# Autodesk Inventor assembly: Shooter-Storage-IntakeAssembly.ver2-1111-2021
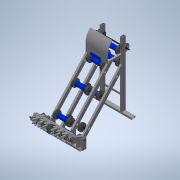
[picture p0: Inventor's stored thumbnail of the model, 180x180]
Saved by Autodesk Inventor 2021 (Build 250183000, 183)
## iProperties
Created: 2020-01-25
Part Number: Shooter-Storage-IntakeAssembly.ver2-1111-2021
Document SubType Name: Assembly
Designer: JMHal
Author: JMHal
## Documents named in this file (6)
- E:\PHRC CADD 2021\PHRC CADD\2020 Infinite Recharge\2021 Infinite Recharge\Chassis\Shooter-Storage-IntakeAssembly.ver2-1111-2021.iam
- E:\PHRC CADD 2021\PHRC CADD\2020 Infinite Recharge\Final Robot Assembly\IntakeAssembly-ver1-1111-2020.iam
- E:\PHRC CADD 2021\PHRC CADD\2020 Infinite Recharge\Shooting\Assemblies\ShooterPrototype-ver2-1111-2019.iam
- E:\PHRC CADD 2021\PHRC CADD\2020 Infinite Recharge\Storage\Assemblies\StorageAssembly.ver4-1111-2020.iam
- E:\PHRC CADD 2021\PHRC CADD\2020 Infinite Recharge\Storage\Assemblies\Roller-ver1-1111-2019.iam
- E:\PHRC CADD 2021\PHRC CADD\2020 Infinite Recharge\Storage\Assemblies\TopRoller-ver1-1111-2019.iam
## Components (12 placed, 5 different names)
1. ShooterPrototype-ver2-1111-2019:1 [sub-assembly] — Mate:1, Flush:10, Mate:2, Mate:3
2. StorageAssembly.ver4-1111-2020:1 [sub-assembly] — Mate:1, Flush:10, Mate:2, Mate:3, Mate:4, Flush:11, Flush:12
3. Roller-ver1-1111-2019:1 [sub-assembly] — Flush:4, Flush:5, Flush:8
4. Roller-ver1-1111-2019:2 [sub-assembly] — Flush:5, Flush:6
5. Roller-ver1-1111-2019:4 [sub-assembly] — Flush:6, Flush:7
6. Roller-ver1-1111-2019:5 [sub-assembly] — Flush:8
7. Roller-ver1-1111-2019:6 [sub-assembly]
8. TopRoller-ver1-1111-2019:1 [sub-assembly] — Flush:3
9. Roller-ver1-1111-2019:7 [sub-assembly] — Flush:9
10. Roller-ver1-1111-2019:8 [sub-assembly] — Flush:3, Flush:4, Flush:9
11. TopRoller-ver1-1111-2019:2 [sub-assembly] — Flush:7
12. IntakeAssembly-ver1-1111-2020:2 [sub-assembly] — Mate:4, Flush:11, Flush:12
## Relationships (14: Flush 10, Mate 4)
- Flush:3: TopRoller-ver1-1111-2019:1 ↔ Roller-ver1-1111-2019:8
- Flush:4: Roller-ver1-1111-2019:1 ↔ Roller-ver1-1111-2019:8
- Flush:5: Roller-ver1-1111-2019:1 ↔ Roller-ver1-1111-2019:2
- Flush:6: Roller-ver1-1111-2019:2 ↔ Roller-ver1-1111-2019:4
- Flush:7: Roller-ver1-1111-2019:4 ↔ TopRoller-ver1-1111-2019:2
- Flush:8: Roller-ver1-1111-2019:1 ↔ Roller-ver1-1111-2019:5
- Flush:9: Roller-ver1-1111-2019:7 ↔ Roller-ver1-1111-2019:8
- Mate:1: ShooterPrototype-ver2-1111-2019:1 ↔ StorageAssembly.ver4-1111-2020:1
- Flush:10: ShooterPrototype-ver2-1111-2019:1 ↔ StorageAssembly.ver4-1111-2020:1
- Mate:2 (100.8888 mm): ShooterPrototype-ver2-1111-2019:1 ↔ StorageAssembly.ver4-1111-2020:1
- Mate:3: ShooterPrototype-ver2-1111-2019:1 ↔ StorageAssembly.ver4-1111-2020:1
- Mate:4: StorageAssembly.ver4-1111-2020:1 ↔ IntakeAssembly-ver1-1111-2020:2
- Flush:11: StorageAssembly.ver4-1111-2020:1 ↔ IntakeAssembly-ver1-1111-2020:2
- Flush:12 (-33.7185 mm): StorageAssembly.ver4-1111-2020:1 ↔ IntakeAssembly-ver1-1111-2020:2
